# Autodesk Inventor assembly: lw_6_сборка_1
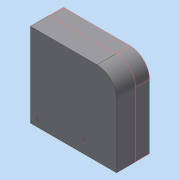
[picture p0: Inventor's stored thumbnail of the model, 180x180]
Saved by Autodesk Inventor 2019 (Build 230136000, 136)
## iProperties
Created: 2021-05-17
Part Number: lw_6_сборка_1
Material: Типовые
Document SubType Name: Assembly
Designer: Kurbatova
Author: Kurbatova
## Documents named in this file (3)
- C:\Users\Kurbatova\source\LW2021\LW_SAPR\Сборки\lw_6_сборка_1.iam
- C:\Users\Kurbatova\source\LW2021\LW_SAPR\Детали\lw_6_part1.ipt
- C:\Users\Kurbatova\source\LW2021\LW_SAPR\Детали\lw_6_part2.ipt
## Components (2 placed, 2 different names)
1. lw_6_part1:1 — Заподлицо:1, Заподлицо:2, Совмещение:1
2. lw_6_part2:1 — Заподлицо:1, Заподлицо:2, Совмещение:1
## Relationships (3: Flush 2, Mate 1)
- Заподлицо:1 [Flush]: lw_6_part1:1 ↔ lw_6_part2:1
- Заподлицо:2 [Flush]: lw_6_part1:1 ↔ lw_6_part2:1
- Совмещение:1 [Mate]: lw_6_part1:1 ↔ lw_6_part2:1
